# Autodesk Inventor assembly: Field Compensation Coils
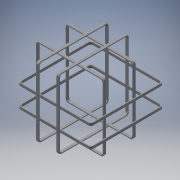
[picture p0: Inventor's stored thumbnail of the model, 180x180]
Saved by Autodesk Inventor 2019 (Build 230136000, 136)
## iProperties
Created: 2021-05-17
Part Number: Field Compensation Coils
Document SubType Name: Assembly
Designer: jamieson-bl
Author: jamieson-bl
## Documents named in this file (4)
- \\Mac\Home\Desktop\DarkPoolDrawings\Field Compensation Coils.iam
- \\Mac\Home\Desktop\DarkPoolDrawings\Coil1or2.ipt
- \\Mac\Home\Desktop\DarkPoolDrawings\Coil3or4.ipt
- \\Mac\Home\Desktop\DarkPoolDrawings\Coil5or6.ipt
## Components (6 placed, 3 different names)
1. Coil1or2:1 — Flush:5, Flush:6, Mate:3, Mate:4
2. Coil1or2:2 — Flush:5, Flush:6, Mate:3, Mate:5, Mate:6, Mate:8
3. Coil3or4:1 — Flush:3, Flush:4, Mate:2
4. Coil3or4:2 — Flush:3, Flush:4, Mate:2, Mate:4, Mate:5, Mate:7, Mate:8
5. Coil5or6:1 — Flush:1, Flush:2, Mate:1, Mate:6, Mate:7
6. Coil5or6:2 — Flush:1, Flush:2, Mate:1
## Relationships (14: Mate 8, Flush 6)
- Flush:1: Coil5or6:1 ↔ Coil5or6:2
- Flush:2: Coil5or6:1 ↔ Coil5or6:2
- Mate:1 (500 mm): Coil5or6:1 ↔ Coil5or6:2
- Flush:3: Coil3or4:1 ↔ Coil3or4:2
- Flush:4: Coil3or4:1 ↔ Coil3or4:2
- Mate:2 (500 mm): Coil3or4:1 ↔ Coil3or4:2
- Flush:5: Coil1or2:1 ↔ Coil1or2:2
- Flush:6: Coil1or2:1 ↔ Coil1or2:2
- Mate:3 (760 mm): Coil1or2:1 ↔ Coil1or2:2
- Mate:4: Coil1or2:1 ↔ Coil3or4:2
- Mate:5 (500 mm): Coil1or2:2 ↔ Coil3or4:2
- Mate:6: Coil1or2:2 ↔ Coil5or6:1
- Mate:7 (500 mm): Coil3or4:2 ↔ Coil5or6:1
- Mate:8 (500 mm): Coil1or2:2 ↔ Coil3or4:2
